# Autodesk Inventor assembly: Pierna_opuesta
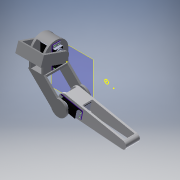
[picture p0: Inventor's stored thumbnail of the model, 180x180]
Saved by Autodesk Inventor 2018 (Build 220112000, 112)
## iProperties
Created: 2020-03-08
Part Number: Pierna_opuesta
Document SubType Name: Assembly
Designer: GonzaloDiaz
Author: GonzaloDiaz
## Documents named in this file (5)
- E:\Universidad\Codigo\Enigma\Diseños\Pierna_opuesta.iam
- E:\Universidad\Codigo\Enigma\Diseños\Femur_opuesto.ipt
- E:\Universidad\Codigo\Enigma\Diseños\SERVOMG996R.ipt
- E:\Universidad\Codigo\Enigma\Diseños\Tibia_opuesta.ipt
- E:\Universidad\Codigo\Enigma\Diseños\Hombro.ipt
## Components (5 placed, 4 different names)
1. Femur_opuesto:1 — Mate:5, Mate:6, Mate:7, Mate:8, Insert:1, Insert:2
2. SERVOMG996R:1 — Mate:5, Mate:6, Mate:7, Mate:8
3. Tibia_opuesta:1 — Mate:9, Mate:10, Mate:11, Insert:2
4. SERVOMG996R:2 — Mate:9, Mate:10, Mate:11
5. Hombro:1 — Insert:1
## Relationships (9: Mate 7, Insert 2)
- Mate:5: Femur_opuesto:1 ↔ SERVOMG996R:1
- Mate:6: Femur_opuesto:1 ↔ SERVOMG996R:1
- Mate:7: Femur_opuesto:1 ↔ SERVOMG996R:1
- Mate:8: Femur_opuesto:1 ↔ SERVOMG996R:1
- Mate:9: Tibia_opuesta:1 ↔ SERVOMG996R:2
- Mate:10: Tibia_opuesta:1 ↔ SERVOMG996R:2
- Mate:11: Tibia_opuesta:1 ↔ SERVOMG996R:2
- Insert:1: Femur_opuesto:1 ↔ Hombro:1
- Insert:2: Femur_opuesto:1 ↔ Tibia_opuesta:1
